# Autodesk Inventor assembly: Collumn
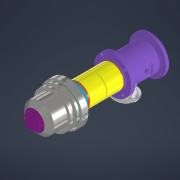
[picture p0: Inventor's stored thumbnail of the model, 180x180]
Saved by Autodesk Inventor 2022 (Build 260153000, 153)
## iProperties
Created: 2022-03-30
Part Number: Collumn
Document SubType Name: Assembly
Designer: Vinicius Miguel
Author: Vinicius Miguel
## Documents named in this file (5)
- C:\ViniFiles\SEM-Mechanical\Collumn.iam
- C:\ViniFiles\SEM-Mechanical\Objective.iam
- C:\ViniFiles\SEM-Mechanical\Condensers.iam
- C:\ViniFiles\SEM-Mechanical\008.ipt
- C:\ViniFiles\SEM-Mechanical\Anode.iam
## Components (4 placed, 4 different names)
1. Objective:1 [sub-assembly] — Mate:1, Flush:1, Flush:2, Mate:4, Mate:8
2. Condensers:1 [sub-assembly] — Mate:2, Mate:5, Mate:9
3. 008:1 — Mate:3, Mate:4, Mate:5, Mate:6
4. Anode:1 [sub-assembly] — Mate:7, Mate:8, Mate:9
## Relationships (11: Mate 9, Flush 2)
- Mate:1: Objective:1
- Flush:1: Objective:1
- Flush:2: Objective:1
- Mate:2: Condensers:1
- Mate:3: 008:1
- Mate:4: Objective:1 ↔ 008:1
- Mate:5: Condensers:1 ↔ 008:1
- Mate:6: 008:1
- Mate:7: Anode:1
- Mate:8: Objective:1 ↔ Anode:1
- Mate:9: Condensers:1 ↔ Anode:1
